# Autodesk Inventor assembly: HDI on BBM
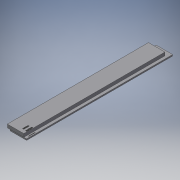
[picture p0: Inventor's stored thumbnail of the model, 180x180]
Saved by Autodesk Inventor 2019.4 (Build 234330000, 330)
## iProperties
Created: 2021-02-08
Part Number: HDI on BBM
Document SubType Name: Assembly
Designer: caleb
Author: caleb
## Documents named in this file (3)
- C:\Users\cfang\Desktop\nebraska-silicon-lab\Hardware\TFPX\module alignment mockup\HDI on BBM.iam
- C:\Users\cfang\Desktop\nebraska-silicon-lab\Hardware\TFPX\module alignment mockup\BBM.ipt
- C:\Users\cfang\Desktop\nebraska-silicon-lab\Hardware\TFPX\module alignment mockup\HDI.ipt
## Components (2 placed, 2 different names)
1. BBM:1 — Mate:1, Angle:1
2. HDI:1 — Mate:1, Angle:1
## Relationships (2: Mate 1, Angle 1)
- Mate:1: BBM:1 ↔ HDI:1
- Angle:1 (0 deg): BBM:1 ↔ HDI:1
